# Autodesk Inventor assembly: OmniWheelGear
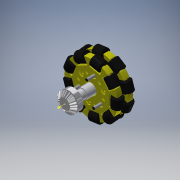
[picture p0: Inventor's stored thumbnail of the model, 180x180]
Saved by Autodesk Inventor 2016 (Build 200138000, 138)
## iProperties
Created: 2017-02-08
Part Number: OmniWheelGear
Document SubType Name: Assembly
Designer: Evan Phil George
Author: Evan Phil George
## Documents named in this file (3)
- C:\Users\Evan Phil George\Desktop\Ball Balancing Robot\TestBenchInventor\SubAssemblies\OmniWheelGear.iam
- C:\Users\Evan Phil George\Desktop\Ball Balancing Robot\TestBenchInventor\SubAssemblies\OmniGear.iam
- C:\Users\Evan Phil George\Desktop\Ball Balancing Robot\TestBenchInventor\OmniWheel\TwoOmniWheelAssembly.iam
## Components (2 placed, 2 different names)
1. TwoOmniWheelAssembly:1 [sub-assembly] — Mate:1, Mate:2, Mate:3
2. OmniGear:1 [sub-assembly] — Mate:1, Mate:2, Mate:3
## Relationships (3: Mate 3)
- Mate:1 (0.1 mm): TwoOmniWheelAssembly:1 ↔ OmniGear:1
- Mate:2 (0.1 mm): TwoOmniWheelAssembly:1 ↔ OmniGear:1
- Mate:3: TwoOmniWheelAssembly:1 ↔ OmniGear:1
